# Autodesk Inventor assembly: DinosaurioEnsmablado
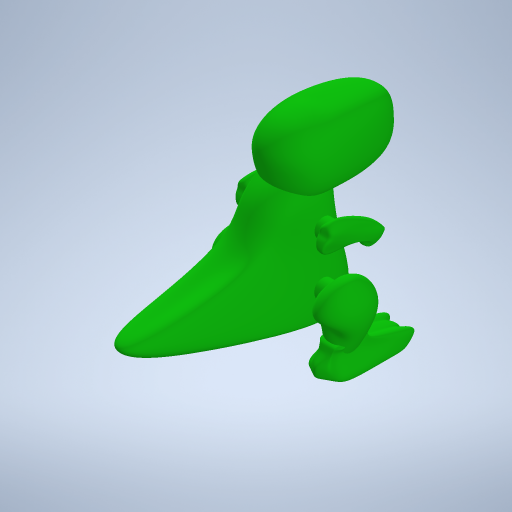
[picture p0: Inventor's stored thumbnail of the model, 512x512]
Saved by Autodesk Inventor 2024.3 (Build 283343000, 343)
## iProperties
Created: 2025-02-09
Part Number: DinosaurioEnsmablado
Document SubType Name: Assembly
Designer: USUARIO
Author: USUARIO
## Documents named in this file (6)
- D:\USUARIO\Documents\Universidad Andres\2024-2\apm\Modelos-Juguetes\Dinosaurio\DinosaurioEnsmablado.iam
- D:\USUARIO\Documents\Universidad Andres\2024-2\apm\Modelos-Juguetes\Dinosaurio\D-Torso.ipt
- D:\USUARIO\Documents\Universidad Andres\2024-2\apm\Modelos-Juguetes\Dinosaurio\D-BrazoDer.ipt
- D:\USUARIO\Documents\Universidad Andres\2024-2\apm\Modelos-Juguetes\Dinosaurio\D-BrazoIzq.ipt
- D:\USUARIO\Documents\Universidad Andres\2024-2\apm\Modelos-Juguetes\Dinosaurio\D-PiernaDer.ipt
- D:\USUARIO\Documents\Universidad Andres\2024-2\apm\Modelos-Juguetes\Dinosaurio\D-PiernaIzq.ipt
## Components (5 placed, 5 different names)
1. D-Torso:1 — Mate:1, Mate:2, Mate:3, Flush:1, Mate:4, Mate:5
2. D-BrazoDer:1 — Mate:1, Mate:2
3. D-BrazoIzq:1 — Mate:3, Flush:1
4. D-PiernaDer:1 — Mate:4
5. D-PiernaIzq:1 — Mate:5, Flush:2
## Relationships (7: Mate 5, Flush 2)
- Mate:1: D-Torso:1 ↔ D-BrazoDer:1
- Mate:2 (7 mm): D-Torso:1 ↔ D-BrazoDer:1
- Mate:3: D-Torso:1 ↔ D-BrazoIzq:1
- Flush:1 (7 mm): D-Torso:1 ↔ D-BrazoIzq:1
- Mate:4: D-Torso:1 ↔ D-PiernaDer:1
- Mate:5: D-Torso:1 ↔ D-PiernaIzq:1
- Flush:2 (-7 mm): D-PiernaIzq:1
